# Autodesk Inventor assembly: hologram display version 2 assembly exploded.ipt
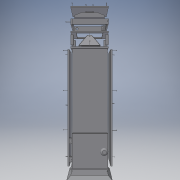
[picture p0: Inventor's stored thumbnail of the model, 180x180]
Saved by Autodesk Inventor 2016 (Build 200138000, 138)
## iProperties
Created: 2017-10-23
Part Number: hologram display version 2 assembly exploded.ipt
Document SubType Name: Assembly
Designer: student
Author: student
## Documents named in this file (15)
- C:\Users\student\Documents\Aaron's Folder\hologram display version 2 assembly exploded.ipt.iam
- C:\Users\student\Documents\Aaron's Folder\base (for assembly).ipt
- C:\Users\student\Documents\Aaron's Folder\support platforms (for assembly).ipt
- C:\Users\student\Documents\Aaron's Folder\side boards (for assembly).ipt
- C:\Users\student\Documents\Aaron's Folder\back board (for assembly).ipt
- C:\Users\student\Documents\Aaron's Folder\front board (for assembly).ipt
- C:\Users\student\Documents\Aaron's Folder\front door (for assembly).ipt
- C:\Users\student\Documents\Aaron's Folder\monitor supports (for assembly).ipt
- C:\Users\student\Documents\Aaron's Folder\monitor frame part1 (for assembly).ipt
- C:\Users\student\Documents\Aaron's Folder\monitor frame part2 (for assembly).ipt
- C:\Users\student\Documents\Aaron's Folder\hologram pyramid (for assembly).ipt
- C:\Users\student\Documents\Aaron's Folder\monitor (for assembly).ipt
- C:\Users\student\Documents\Aaron's Folder\screws (for assembly).ipt
- C:\Users\student\Documents\Aaron's Folder\hinges (for assembly).ipt
- C:\Users\student\Documents\Aaron's Folder\VESA mount.ipt
## Components (70 placed, 14 different names)
1. base (for assembly):1 — Rigid:1
2. support platforms (for assembly):1 — Rigid:1, Rigid:19
3. side boards (for assembly):1 — Rigid:18
4. side boards (for assembly):2 — Rigid:18
5. support platforms (for assembly):2 — Rigid:19, Rigid:20, Rigid:21, Rigid:22, Rigid:24, Rigid:33
6. back board (for assembly):1 — Rigid:15, Rigid:16
7. front board (for assembly):1 — Rigid:16
8. front door (for assembly):1 — Rigid:15
9. monitor supports (for assembly):2 — Rigid:21
10. monitor supports (for assembly):3 — Rigid:20, Rigid:25
11. monitor supports (for assembly):4 — Rigid:22
12. hologram pyramid (for assembly):1 — Rigid:24
13. monitor frame part1 (for assembly):1 — Rigid:25, Rigid:27
14. monitor frame part2 (for assembly):1
15. monitor (for assembly):1 — Rigid:27, Rigid:30
16. support platforms (for assembly):3 — Rotational:1, Rotational:2, Rotational:4, Rotational:5
17. screws (for assembly):5
18. screws (for assembly):6
19. screws (for assembly):7
20. screws (for assembly):8
21. screws (for assembly):9
22. screws (for assembly):10
23. screws (for assembly):11
24. screws (for assembly):12
25. screws (for assembly):13
26. screws (for assembly):14
27. screws (for assembly):15
28. screws (for assembly):16
29. screws (for assembly):17
30. screws (for assembly):18
31. screws (for assembly):19
32. screws (for assembly):20
33. screws (for assembly):21
34. screws (for assembly):22
35. screws (for assembly):23
36. screws (for assembly):24
37. screws (for assembly):26
38. screws (for assembly):27
39. screws (for assembly):28
40. screws (for assembly):29
41. screws (for assembly):30
42. screws (for assembly):31
43. screws (for assembly):32
44. screws (for assembly):33
45. screws (for assembly):34
46. screws (for assembly):35
47. screws (for assembly):36
48. screws (for assembly):37
49. screws (for assembly):38
50. screws (for assembly):39
51. screws (for assembly):40
52. screws (for assembly):41
53. screws (for assembly):42
54. screws (for assembly):43
55. screws (for assembly):44
56. screws (for assembly):45
57. screws (for assembly):46
58. hinges (for assembly):1
59. hinges (for assembly):2
60. screws (for assembly):47
61. screws (for assembly):48
62. hinges (for assembly):3
63. VESA mount:1 — Rigid:30, Rigid:31
64. VESA mount:2 — Rigid:31, Rigid:32
65. VESA mount:3 — Rigid:32
66. monitor supports (for assembly):5 — Rigid:33
67. screws (for assembly):49 — Rotational:1
68. screws (for assembly):50 — Rotational:2
69. screws (for assembly):52 — Rotational:4
70. screws (for assembly):53 — Rotational:5
## Relationships (19: WeldJoint 15, RevoluteJoint 4)
- Rigid:1 [WeldJoint] (76.2 mm): base (for assembly):1 ↔ support platforms (for assembly):1
- Rigid:15 [WeldJoint] (508 mm): back board (for assembly):1 ↔ front door (for assembly):1
- Rigid:16 [WeldJoint] (457.2 mm): back board (for assembly):1 ↔ front board (for assembly):1
- Rigid:18 [WeldJoint] (558.8 mm): side boards (for assembly):1 ↔ side boards (for assembly):2
- Rigid:19 [WeldJoint] (1625.6 mm): support platforms (for assembly):1 ↔ support platforms (for assembly):2
- Rigid:20 [WeldJoint] (25.4 mm): support platforms (for assembly):2 ↔ monitor supports (for assembly):3
- Rigid:21 [WeldJoint] (25.4 mm): support platforms (for assembly):2 ↔ monitor supports (for assembly):2
- Rigid:22 [WeldJoint] (25.4 mm): support platforms (for assembly):2 ↔ monitor supports (for assembly):4
- Rigid:24 [WeldJoint] (190.5 mm): support platforms (for assembly):2 ↔ hologram pyramid (for assembly):1
- Rigid:25 [WeldJoint] (25.4 mm): monitor supports (for assembly):3 ↔ monitor frame part1 (for assembly):1
- Rigid:27 [WeldJoint] (198.12 mm): monitor frame part1 (for assembly):1 ↔ monitor (for assembly):1
- Rigid:30 [WeldJoint] (12.7 mm): monitor (for assembly):1 ↔ VESA mount:1
- Rigid:31 [WeldJoint] (12.7 mm): VESA mount:1 ↔ VESA mount:2
- Rigid:32 [WeldJoint] (12.7 mm): VESA mount:2 ↔ VESA mount:3
- Rigid:33 [WeldJoint] (25.4 mm): support platforms (for assembly):2 ↔ monitor supports (for assembly):5
- Rotational:1 [RevoluteJoint] (7.62 mm): support platforms (for assembly):3 ↔ screws (for assembly):49
- Rotational:2 [RevoluteJoint] (7.62 mm): support platforms (for assembly):3 ↔ screws (for assembly):50
- Rotational:4 [RevoluteJoint] (7.62 mm): support platforms (for assembly):3 ↔ screws (for assembly):52
- Rotational:5 [RevoluteJoint] (7.62 mm): support platforms (for assembly):3 ↔ screws (for assembly):53
